# Autodesk Inventor assembly: Assembly
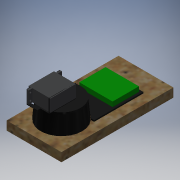
[picture p0: Inventor's stored thumbnail of the model, 180x180]
Saved by Autodesk Inventor 2017 (Build 210142000, 142)
## iProperties
Created: 2018-10-14
Part Number: Assembly
Document SubType Name: Assembly
Designer: Cameron
Author: Cameron
## Documents named in this file (8)
- C:\Users\Cameron\Desktop\Robotics\Assembly.iam
- C:\Users\Cameron\Desktop\Robotics\Base.ipt
- C:\Users\Cameron\Desktop\Robotics\Electronics Plate.ipt
- C:\Users\Cameron\Desktop\Robotics\Motherboard.ipt
- C:\Users\Cameron\Desktop\Robotics\Rotating Top.ipt
- C:\Users\Cameron\Desktop\Robotics\Shoulder Plate.ipt
- C:\Users\Cameron\Desktop\Robotics\Shoulder Servo.ipt
- C:\Users\Cameron\Desktop\Robotics\Wooden Base.ipt
## Components (7 placed, 7 different names)
1. Base:1 — Mate:1, Mate:2, Mate:3, Mate:5, Mate:7, Mate:8
2. Electronics Plate:1 — Mate:4, Mate:5, Mate:6, Flush:1, Flush:2
3. Motherboard:1 — Mate:6, Flush:1, Flush:2
4. Rotating Top:1 — Mate:7, Mate:8, Mate:9, Mate:10, Mate:11
5. Shoulder Plate:1 — Mate:9, Mate:10, Mate:11, Mate:12, Mate:13, Mate:14
6. Shoulder Servo:1 — Mate:12, Mate:13, Mate:14
7. Wooden Base:1 — Mate:1, Mate:2, Mate:3, Mate:4
## Relationships (16: Mate 14, Flush 2)
- Mate:1: Base:1 ↔ Wooden Base:1
- Mate:2 (-65 mm): Base:1 ↔ Wooden Base:1
- Mate:3 (-65 mm): Base:1 ↔ Wooden Base:1
- Mate:4: Electronics Plate:1 ↔ Wooden Base:1
- Mate:5: Base:1 ↔ Electronics Plate:1
- Mate:6: Electronics Plate:1 ↔ Motherboard:1
- Flush:1 (5 mm): Electronics Plate:1 ↔ Motherboard:1
- Flush:2 (-5 mm): Electronics Plate:1 ↔ Motherboard:1
- Mate:7: Base:1 ↔ Rotating Top:1
- Mate:8: Base:1 ↔ Rotating Top:1
- Mate:9: Rotating Top:1 ↔ Shoulder Plate:1
- Mate:10 (-20 mm): Rotating Top:1 ↔ Shoulder Plate:1
- Mate:11 (-20 mm): Rotating Top:1 ↔ Shoulder Plate:1
- Mate:12: Shoulder Plate:1 ↔ Shoulder Servo:1
- Mate:13: Shoulder Plate:1 ↔ Shoulder Servo:1
- Mate:14: Shoulder Plate:1 ↔ Shoulder Servo:1
